# Autodesk Inventor assembly: KP08
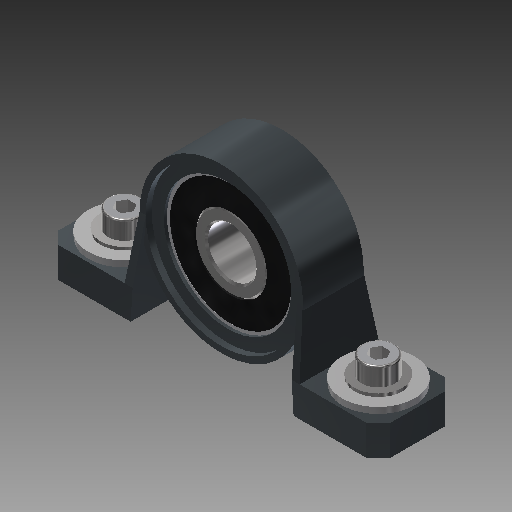
[picture p0: Inventor's stored thumbnail of the model, 512x512]
Saved by Autodesk Inventor 2017 SP1 (Build 210196100, 196)
## iProperties
Part Number: KP08
Material: Generisch
Document SubType Name: Assembly
Designer: Till
Author: Till
## Documents named in this file (7)
- C:\Users\Till\Dropbox\DIY\CAD\KP08\KP08.iam
- C:\Users\Till\Dropbox\DIY\CAD\KP08\Huelse.ipt
- C:\Users\Till\Dropbox\DIY\CAD\KP08\dichtung.ipt
- C:\Users\Till\Dropbox\DIY\CAD\KP08\außenlager.ipt
- C:\Users\Till\Dropbox\DIY\CAD\KP08\lagerblock.ipt
- C:\Users\Till\Dropbox\DIY\CoreBot\CAD Parts\unterlegscheibe_iso_7093-4-140_hv.ipt
- C:\Users\Till\Dropbox\DIY\CoreBot\M3 x 10.ipt
## Components (8 placed, 6 different names)
1. Huelse:1 — Passend:1, Fluchtend:1
2. dichtung:1 — Passend:1, Fluchtend:1, Passend:2, Fluchtend:2
3. außenlager:1 — Passend:2, Fluchtend:2, Passend:3, Passend:4, Fluchtend:3
4. lagerblock:1 — Passend:3, Passend:4, Fluchtend:3, Passend:5, Passend:6, Passend:7, Passend:12, Passend:13, Passend:14, Passend:15
5. unterlegscheibe_iso_7093-4-140_hv:1 — Passend:10, Passend:11, Passend:13
6. unterlegscheibe_iso_7093-4-140_hv:2 — Passend:8, Passend:9, Passend:15
7. M3 x 10:1 — Passend:8, Passend:9, Passend:14
8. M3 x 10:2 — Passend:10, Passend:11, Passend:12
## Relationships (18: Mate 15, Flush 3)
- Passend:1 [Mate]: Huelse:1 ↔ dichtung:1
- Fluchtend:1 [Flush]: Huelse:1 ↔ dichtung:1
- Passend:2 [Mate]: dichtung:1 ↔ außenlager:1
- Fluchtend:2 [Flush]: dichtung:1 ↔ außenlager:1
- Passend:3 [Mate] (10.5 mm): außenlager:1 ↔ lagerblock:1
- Passend:4 [Mate]: außenlager:1 ↔ lagerblock:1
- Fluchtend:3 [Flush] (-0.5 mm): außenlager:1 ↔ lagerblock:1
- Passend:5 [Mate]: lagerblock:1
- Passend:6 [Mate]: lagerblock:1
- Passend:7 [Mate]: lagerblock:1
- Passend:8 [Mate]: unterlegscheibe_iso_7093-4-140_hv:2 ↔ M3 x 10:1
- Passend:9 [Mate]: unterlegscheibe_iso_7093-4-140_hv:2 ↔ M3 x 10:1
- Passend:10 [Mate]: unterlegscheibe_iso_7093-4-140_hv:1 ↔ M3 x 10:2
- Passend:11 [Mate]: unterlegscheibe_iso_7093-4-140_hv:1 ↔ M3 x 10:2
- Passend:12 [Mate]: lagerblock:1 ↔ M3 x 10:2
- Passend:13 [Mate]: lagerblock:1 ↔ unterlegscheibe_iso_7093-4-140_hv:1
- Passend:14 [Mate]: lagerblock:1 ↔ M3 x 10:1
- Passend:15 [Mate]: lagerblock:1 ↔ unterlegscheibe_iso_7093-4-140_hv:2
